# Autodesk Inventor assembly: Gantry1
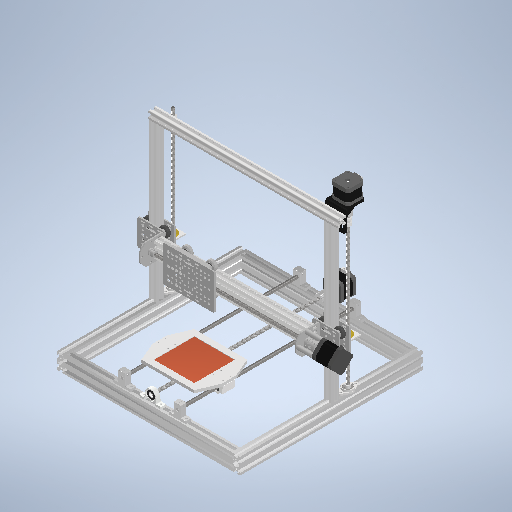
[picture p0: Inventor's stored thumbnail of the model, 512x512]
Saved by Autodesk Inventor 2025.2 (Build 292293000, 293)
## iProperties
Created: 2025-05-31
Part Number: Gantry1
Document SubType Name: Assembly
Designer: Simon
Author: Simon
## Documents named in this file (35)
- C:\Users\Simon\Projects\Hydrogel-3D-Printer\Hardware\Bioprinter Machine Design\Gantry Concept 1\Gantry1.iam
- C:\Users\Simon\Projects\Hydrogel-3D-Printer\Hardware\Bioprinter Machine Design\Gantry Concept 1\SteelShaft_444mm.ipt
- C:\Users\Simon\Projects\Hydrogel-3D-Printer\Hardware\Bioprinter Machine Design\PartsFolder\SK8_LinearShaftSupport.ipt
- C:\Users\Simon\Projects\Hydrogel-3D-Printer\Hardware\Bioprinter Machine Design\PartsFolder\PeltierTEC1_12706.ipt
- C:\Users\Simon\Projects\Hydrogel-3D-Printer\Hardware\Bioprinter Machine Design\PartsFolder\SC8UU\SC8UU.iam
- C:\Users\Simon\Projects\Hydrogel-3D-Printer\Hardware\Bioprinter Machine Design\Gantry Concept 1\BedPlate.ipt
- C:\Users\Simon\Projects\Hydrogel-3D-Printer\Hardware\Bioprinter Machine Design\Gantry Concept 1\BedHousingFrame.ipt
- C:\Users\Simon\Projects\Hydrogel-3D-Printer\Hardware\Bioprinter Machine Design\Gantry Concept 1\2040_AluminimProfile_450.ipt
- C:\Users\Simon\Projects\Hydrogel-3D-Printer\Hardware\Bioprinter Machine Design\Gantry Concept 1\2040_AluminimProfile_410.ipt
- C:\Users\Simon\Projects\Hydrogel-3D-Printer\Hardware\Bioprinter Machine Design\PartsFolder\bracket nema 17.ipt
- C:\Users\Simon\Projects\Hydrogel-3D-Printer\Hardware\Bioprinter Machine Design\Gantry Concept 1\2020_AluminiumProfile_380.ipt
- C:\Users\Simon\Projects\Hydrogel-3D-Printer\Hardware\Bioprinter Machine Design\PartsFolder\Pillow Block Bearing 1\Zinc Alloy Pillow Block Flange Bearing KFL08 ID-8mm.iam
- C:\Users\Simon\Projects\Hydrogel-3D-Printer\Hardware\Bioprinter Machine Design\Gantry Concept 1\TR8x8-4_LeadScrew_385mm.ipt
- C:\Users\Simon\Projects\Hydrogel-3D-Printer\Hardware\Bioprinter Machine Design\PartsFolder\Stepper_17HS4401.ipt
- C:\Users\Simon\Projects\Hydrogel-3D-Printer\Hardware\Bioprinter Machine Design\PartsFolder\GT2_20T_8.ipt
- C:\Users\Simon\Projects\Hydrogel-3D-Printer\Hardware\Bioprinter Machine Design\PartsFolder\Flexible Coupling 5,8.ipt
- C:\Users\Simon\Projects\Hydrogel-3D-Printer\Hardware\Bioprinter Machine Design\Gantry Concept 1\2020_AluminiumProfile_465.ipt
- C:\Users\Simon\Projects\Hydrogel-3D-Printer\Hardware\Bioprinter Machine Design\PartsFolder\TR8x8-4_Nut.ipt
- C:\Users\Simon\Projects\Hydrogel-3D-Printer\Hardware\Bioprinter Machine Design\PartsFolder\Carriage Plate v1.ipt
- C:\Users\Simon\Projects\Hydrogel-3D-Printer\Hardware\Bioprinter Machine Design\PartsFolder\Spacer v2.ipt
- C:\Users\Simon\Projects\Hydrogel-3D-Printer\Hardware\Bioprinter Machine Design\PartsFolder\POM Wheel v2.ipt
- C:\Users\Simon\Projects\Hydrogel-3D-Printer\Hardware\Bioprinter Machine Design\Gantry Concept 1\Lead Screw Driven Actuator (Horizontal)\2040 Al Extrusion - Upper Middle Part (380mm).ipt
- C:\Users\Simon\Projects\Hydrogel-3D-Printer\Hardware\Bioprinter Machine Design\Gantry Concept 1\Lead Screw Driven Actuator (Horizontal)\Threaded Rod Plate Nema 17.ipt
- C:\Users\Simon\Projects\Hydrogel-3D-Printer\Hardware\Bioprinter Machine Design\Gantry Concept 1\Lead Screw Driven Actuator (Horizontal)\Nema 17 Stepper Motor.ipt
- C:\Users\Simon\Projects\Hydrogel-3D-Printer\Hardware\Bioprinter Machine Design\Gantry Concept 1\Lead Screw Driven Actuator (Horizontal)\Aluminum Spacer 1.5in.ipt
- C:\Users\Simon\Projects\Hydrogel-3D-Printer\Hardware\Bioprinter Machine Design\Gantry Concept 1\Lead Screw Driven Actuator (Horizontal)\Flexible Coupling 5mm x 8mm.ipt
- C:\Users\Simon\Projects\Hydrogel-3D-Printer\Hardware\Bioprinter Machine Design\Gantry Concept 1\Lead Screw Driven Actuator (Horizontal)\Lead Screw D8-P2-L400 (ACME).ipt
- C:\Users\Simon\Projects\Hydrogel-3D-Printer\Hardware\Bioprinter Machine Design\Gantry Concept 1\Lead Screw Driven Actuator (Horizontal)\Lead Screw Accessories\Ball Bearing 8 x 16 x 5.ipt
- C:\Users\Simon\Projects\Hydrogel-3D-Printer\Hardware\Bioprinter Machine Design\Gantry Concept 1\Lead Screw Driven Actuator (Horizontal)\Lead Screw Accessories\Lock Collar 8mm.ipt
- C:\Users\Simon\Projects\Hydrogel-3D-Printer\Hardware\Bioprinter Machine Design\Gantry Concept 1\Lead Screw Driven Actuator (Horizontal)\Lead Screw Accessories\Shim Washer 8mm.ipt
- C:\Users\Simon\Projects\Hydrogel-3D-Printer\Hardware\Bioprinter Machine Design\Gantry Concept 1\Lead Screw Driven Actuator (Horizontal)\V-Slot Gantry Kit Universal (for lead screw setup)\Gantry Kit (Horizontal).iam
- C:\Users\Simon\Projects\Hydrogel-3D-Printer\Hardware\Bioprinter Machine Design\Gantry Concept 1\Leadnut Attachment.ipt
- C:\Users\Simon\Projects\Hydrogel-3D-Printer\Hardware\Bioprinter Machine Design\PartsFolder\Pillow Block Bearing 2\KP08_2.iam
- C:\Users\Simon\Projects\Hydrogel-3D-Printer\Hardware\Bioprinter Machine Design\PartsFolder\Nema 17 Flat Mount.ipt
- C:\Users\Simon\Projects\Hydrogel-3D-Printer\Hardware\Bioprinter Machine Design\Gantry Concept 1\TR8x8-4_LeadScrew_420.ipt
## Components (80 placed, 34 different names)
1. SteelShaft_444mm:1 — Mate:1, Mate:3, Flush:1, Flush:4, Mate:5
2. SteelShaft_444mm:2 — Mate:2, Mate:4, Flush:2, Flush:3, Mate:6
3. SK8_LinearShaftSupport:1 — Mate:1, Flush:1, Flush:5, Flush:6, Mate:26
4. SK8_LinearShaftSupport:2 — Mate:2, Flush:2, Flush:5, Flush:6, Mate:23, Flush:19, Flush:45, Flush:47
5. SK8_LinearShaftSupport:3 — Mate:3, Flush:4, Mate:25
6. SK8_LinearShaftSupport:4 — Mate:4, Flush:3, Mate:24
7. PeltierTEC1_12706:1 — Mate:7, Flush:7, Flush:8
8. SC8UU:1 [sub-assembly] — Mate:5, Mate:11, Flush:9, Flush:11, Flush:12
9. SC8UU:2 [sub-assembly] — Mate:6, Flush:10, Mate:12, Flush:11
10. BedPlate:1 — Mate:7, Flush:7, Flush:8, Mate:8, Mate:9, Mate:10
11. BedHousingFrame:1 — Mate:8, Mate:9, Mate:10, Mate:11, Flush:9, Flush:10, Mate:12, Flush:12
12. 2040_AluminimProfile_450:1 — Mate:17, Flush:13, Flush:14, Mate:19, Flush:17, Flush:18, Mate:21, Mate:27, Flush:21, Mate:30, Mate:32
13. 2040_AluminimProfile_450:2 — Mate:18, Flush:15, Flush:16, Mate:23, Mate:24, Mate:28, Flush:20, Mate:29, Mate:31, Flush:45, Flush:46, Flush:48
14. 2040_AluminimProfile_410:1 — Mate:17, Flush:13, Flush:14, Mate:18, Flush:15, Flush:16, Mate:20, Mate:26, Flush:19, Mate:165
15. 2040_AluminimProfile_410:2 — Mate:19, Flush:17, Flush:18, Mate:22, Mate:25, Mate:167, Angle:3
16. bracket nema 17:1 — Mate:36, Mate:37, Mate:40, Angle:1
17. 2020_AluminiumProfile_380:1 — Mate:28, Flush:20, Flush:22, Flush:33, Flush:34, Flush:46
18. 2020_AluminiumProfile_380:2 — Mate:27, Flush:21, Flush:22, Mate:35, Flush:25, Flush:26, Flush:31, Flush:32
19. Zinc Alloy Pillow Block Flange Bearing KFL08 ID-8mm:1 [sub-assembly] — Mate:29, Mate:31, Flush:23, Mate:33, Flush:28
20. Zinc Alloy Pillow Block Flange Bearing KFL08 ID-8mm:2 [sub-assembly] — Mate:30, Mate:32, Flush:23, Mate:34
21. TR8x8-4_LeadScrew_385mm:1 — Mate:33, Flush:24, Mate:36, Mate:38, Flush:28, Mate:41, Mate:42, Mate:45
22. TR8x8-4_LeadScrew_385mm:2 — Mate:34, Flush:24, Mate:43, Mate:46
23. Stepper_17HS4401:1 — Mate:38, Mate:39, Flush:27, Mate:40, Mate:41, Angle:1
24. GT2_20T_8:1 — Mate:42, Flush:29, Mate:44
25. GT2_20T_8:2 — Mate:43, Flush:29
26. Flexible Coupling 5,8:1 — Mate:39, Flush:27, Mate:44
27. 2020_AluminiumProfile_465:1 — Mate:35, Flush:25, Flush:26, Mate:37
28. TR8x8-4_Nut:1 — Mate:45, Flush:30, Mate:164
29. TR8x8-4_Nut:2 — Mate:46, Flush:30
30. Carriage Plate v1:1 — Mate:71, Mate:72, Mate:73, Mate:158, Mate:159, Mate:160
31. Carriage Plate v1:2 — Mate:47, Mate:48, Mate:49, Mate:50, Mate:51, Mate:52, Mate:53, Mate:54, Flush:32, Flush:35, Mate:157, Flush:43, Flush:44
32. Spacer v2:1 — Mate:49, Mate:54, Mate:58, Mate:66
33. Spacer v2:2 — Mate:47, Mate:51, Mate:56, Mate:64
34. Spacer v2:3 — Mate:50, Mate:53, Mate:57, Mate:65
35. Spacer v2:4 — Mate:48, Mate:52, Mate:55, Mate:63
36. Spacer v2:5 — Mate:59, Mate:67
37. Spacer v2:6 — Mate:61, Mate:68, Mate:71
38. Spacer v2:7 — Mate:62, Mate:69
39. Spacer v2:8 — Mate:60, Mate:70, Mate:72, Mate:73
40. POM Wheel v2:1 — Mate:58, Mate:60, Mate:66, Mate:70
41. POM Wheel v2:2 — Mate:57, Mate:62, Mate:65, Mate:69
42. POM Wheel v2:3 — Mate:56, Mate:59, Mate:64, Mate:67
43. POM Wheel v2:4 — Mate:55, Mate:61, Mate:63, Mate:68, Flush:31
44. Carriage Plate v1:5 — Mate:161, Mate:162, Mate:163
45. Carriage Plate v1:6 — Flush:34, Flush:35
46. Spacer v2:17
47. Spacer v2:18
48. Spacer v2:19
49. Spacer v2:20
50. Spacer v2:21
51. Spacer v2:22
52. Spacer v2:23
53. Spacer v2:24
54. POM Wheel v2:9
55. POM Wheel v2:10
56. POM Wheel v2:11 — Flush:33
57. POM Wheel v2:12
58. 2040 Al Extrusion - Upper Middle Part (380mm):1
59. Threaded Rod Plate Nema 17:1 — Mate:157, Flush:43, Flush:44
60. Threaded Rod Plate Nema 17:2
61. Nema 17 Stepper Motor:1
62. Aluminum Spacer 1.5in:1
63. Aluminum Spacer 1.5in:2
64. Aluminum Spacer 1.5in:3
65. Flexible Coupling 5mm x 8mm:1
66. Lead Screw D8-P2-L400 (ACME):1
67. Ball Bearing 8 x 16 x 5:1
68. Ball Bearing 8 x 16 x 5:2
69. Lock Collar 8mm:1
70. Lock Collar 8mm:2
71. Shim Washer 8mm:1
72. Shim Washer 8mm:2
73. Gantry Kit (Horizontal):1 [sub-assembly]
74. Leadnut Attachment:1 — Mate:158, Mate:159, Mate:160
75. Leadnut Attachment:2 — Mate:161, Mate:162, Mate:163, Mate:164
76. Stepper_17HS4401:2 — Mate:168, Angle:2, Mate:169, Mate:170, Flush:49, Mate:172
77. KP08_2:1 [sub-assembly] — Mate:165, Flush:47, Flush:48, Mate:166
78. Nema 17 Flat Mount:1 — Mate:166, Mate:167, Mate:168, Angle:2, Angle:3, Mate:169
79. Flexible Coupling 5,8:2 — Mate:170, Flush:49, Mate:171
80. TR8x8-4_LeadScrew_420:1 — Mate:171, Mate:172
## Relationships (194: Mate 141, Flush 49, Angle 3, RelateRotateTranslate 1)
- Mate:1: SteelShaft_444mm:1 ↔ SK8_LinearShaftSupport:1
- Mate:2: SteelShaft_444mm:2 ↔ SK8_LinearShaftSupport:2
- Mate:3: SteelShaft_444mm:1 ↔ SK8_LinearShaftSupport:3
- Mate:4: SteelShaft_444mm:2 ↔ SK8_LinearShaftSupport:4
- Flush:1: SteelShaft_444mm:1 ↔ SK8_LinearShaftSupport:1
- Flush:2: SteelShaft_444mm:2 ↔ SK8_LinearShaftSupport:2
- Flush:3: SteelShaft_444mm:2 ↔ SK8_LinearShaftSupport:4
- Flush:4: SteelShaft_444mm:1 ↔ SK8_LinearShaftSupport:3
- Flush:5: SK8_LinearShaftSupport:1 ↔ SK8_LinearShaftSupport:2
- Flush:6: SK8_LinearShaftSupport:1 ↔ SK8_LinearShaftSupport:2
- Mate:5: SteelShaft_444mm:1 ↔ SC8UU:1
- Mate:6: SteelShaft_444mm:2 ↔ SC8UU:2
- Mate:7: PeltierTEC1_12706:1 ↔ BedPlate:1
- Flush:7 (-30 mm): PeltierTEC1_12706:1 ↔ BedPlate:1
- Flush:8 (30 mm): PeltierTEC1_12706:1 ↔ BedPlate:1
- Mate:8: BedPlate:1 ↔ BedHousingFrame:1
- Mate:9: BedPlate:1 ↔ BedHousingFrame:1
- Mate:10: BedPlate:1 ↔ BedHousingFrame:1
- Mate:11: SC8UU:1 ↔ BedHousingFrame:1
- Flush:9: SC8UU:1 ↔ BedHousingFrame:1
- Flush:10: SC8UU:2 ↔ BedHousingFrame:1
- Mate:12: SC8UU:2 ↔ BedHousingFrame:1
- Flush:11: SC8UU:1 ↔ SC8UU:2
- Flush:12 (50 mm): SC8UU:1 ↔ BedHousingFrame:1
- Mate:17: 2040_AluminimProfile_450:1 ↔ 2040_AluminimProfile_410:1
- Flush:13: 2040_AluminimProfile_450:1 ↔ 2040_AluminimProfile_410:1
- Flush:14: 2040_AluminimProfile_450:1 ↔ 2040_AluminimProfile_410:1
- Mate:18: 2040_AluminimProfile_450:2 ↔ 2040_AluminimProfile_410:1
- Flush:15: 2040_AluminimProfile_450:2 ↔ 2040_AluminimProfile_410:1
- Flush:16: 2040_AluminimProfile_450:2 ↔ 2040_AluminimProfile_410:1
- Mate:19: 2040_AluminimProfile_450:1 ↔ 2040_AluminimProfile_410:2
- Flush:17: 2040_AluminimProfile_450:1 ↔ 2040_AluminimProfile_410:2
- Flush:18: 2040_AluminimProfile_450:1 ↔ 2040_AluminimProfile_410:2
- Mate:20: 2040_AluminimProfile_410:1
- Mate:21: 2040_AluminimProfile_450:1
- Mate:22: 2040_AluminimProfile_410:2
- Mate:23: SK8_LinearShaftSupport:2 ↔ 2040_AluminimProfile_450:2
- Mate:24: SK8_LinearShaftSupport:4 ↔ 2040_AluminimProfile_450:2
- Mate:25: SK8_LinearShaftSupport:3 ↔ 2040_AluminimProfile_410:2
- Mate:26: SK8_LinearShaftSupport:1 ↔ 2040_AluminimProfile_410:1
- Flush:19 (3 mm): SK8_LinearShaftSupport:2 ↔ 2040_AluminimProfile_410:1
- Mate:27: 2040_AluminimProfile_450:1 ↔ 2020_AluminiumProfile_380:2
- Mate:28: 2040_AluminimProfile_450:2 ↔ 2020_AluminiumProfile_380:1
- Flush:20: 2040_AluminimProfile_450:2 ↔ 2020_AluminiumProfile_380:1
- Flush:21: 2040_AluminimProfile_450:1 ↔ 2020_AluminiumProfile_380:2
- Flush:22: 2020_AluminiumProfile_380:1 ↔ 2020_AluminiumProfile_380:2
- Mate:29: 2040_AluminimProfile_450:2 ↔ Zinc Alloy Pillow Block Flange Bearing KFL08 ID-8mm:1
- Mate:30: 2040_AluminimProfile_450:1 ↔ Zinc Alloy Pillow Block Flange Bearing KFL08 ID-8mm:2
- Mate:31: 2040_AluminimProfile_450:2 ↔ Zinc Alloy Pillow Block Flange Bearing KFL08 ID-8mm:1
- Mate:32: 2040_AluminimProfile_450:1 ↔ Zinc Alloy Pillow Block Flange Bearing KFL08 ID-8mm:2
- Flush:23: Zinc Alloy Pillow Block Flange Bearing KFL08 ID-8mm:1 ↔ Zinc Alloy Pillow Block Flange Bearing KFL08 ID-8mm:2
- Mate:33: Zinc Alloy Pillow Block Flange Bearing KFL08 ID-8mm:1 ↔ TR8x8-4_LeadScrew_385mm:1
- Mate:34: Zinc Alloy Pillow Block Flange Bearing KFL08 ID-8mm:2 ↔ TR8x8-4_LeadScrew_385mm:2
- Flush:24: TR8x8-4_LeadScrew_385mm:1 ↔ TR8x8-4_LeadScrew_385mm:2
- Mate:35: 2020_AluminiumProfile_380:2 ↔ 2020_AluminiumProfile_465:1
- Flush:25: 2020_AluminiumProfile_380:2 ↔ 2020_AluminiumProfile_465:1
- Flush:26: 2020_AluminiumProfile_380:2 ↔ 2020_AluminiumProfile_465:1
- Mate:36: bracket nema 17:1 ↔ TR8x8-4_LeadScrew_385mm:1
- Mate:37: bracket nema 17:1 ↔ 2020_AluminiumProfile_465:1
- Mate:38: TR8x8-4_LeadScrew_385mm:1 ↔ Stepper_17HS4401:1
- Mate:39: Stepper_17HS4401:1 ↔ Flexible Coupling 5,8:1
- Flush:27 (5 mm): Stepper_17HS4401:1 ↔ Flexible Coupling 5,8:1
- Mate:40: bracket nema 17:1 ↔ Stepper_17HS4401:1
- Flush:28: Zinc Alloy Pillow Block Flange Bearing KFL08 ID-8mm:1 ↔ TR8x8-4_LeadScrew_385mm:1
- Mate:41: TR8x8-4_LeadScrew_385mm:1 ↔ Stepper_17HS4401:1
- Angle:1 (0 deg): bracket nema 17:1 ↔ Stepper_17HS4401:1
- Mate:42: TR8x8-4_LeadScrew_385mm:1 ↔ GT2_20T_8:1
- Mate:43: TR8x8-4_LeadScrew_385mm:2 ↔ GT2_20T_8:2
- Flush:29: GT2_20T_8:1 ↔ GT2_20T_8:2
- Mate:44 (5 mm): GT2_20T_8:1 ↔ Flexible Coupling 5,8:1
- Mate:45: TR8x8-4_LeadScrew_385mm:1 ↔ TR8x8-4_Nut:1
- Mate:46: TR8x8-4_LeadScrew_385mm:2 ↔ TR8x8-4_Nut:2
- Flush:30: TR8x8-4_Nut:1 ↔ TR8x8-4_Nut:2
- Mate:47: Carriage Plate v1:2 ↔ Spacer v2:2
- Mate:48: Carriage Plate v1:2 ↔ Spacer v2:4
- Mate:49: Carriage Plate v1:2 ↔ Spacer v2:1
- Mate:50: Carriage Plate v1:2 ↔ Spacer v2:3
- Mate:51: Carriage Plate v1:2 ↔ Spacer v2:2
- Mate:52: Carriage Plate v1:2 ↔ Spacer v2:4
- Mate:53: Carriage Plate v1:2 ↔ Spacer v2:3
- Mate:54: Carriage Plate v1:2 ↔ Spacer v2:1
- Mate:55: Spacer v2:4 ↔ POM Wheel v2:4
- Mate:56: Spacer v2:2 ↔ POM Wheel v2:3
- Mate:57: Spacer v2:3 ↔ POM Wheel v2:2
- Mate:58: Spacer v2:1 ↔ POM Wheel v2:1
- Mate:59: Spacer v2:5 ↔ POM Wheel v2:3
- Mate:60: Spacer v2:8 ↔ POM Wheel v2:1
- Mate:61: Spacer v2:6 ↔ POM Wheel v2:4
- Mate:62: Spacer v2:7 ↔ POM Wheel v2:2
- Mate:63: Spacer v2:4 ↔ POM Wheel v2:4
- Mate:64: Spacer v2:2 ↔ POM Wheel v2:3
- Mate:65: Spacer v2:3 ↔ POM Wheel v2:2
- Mate:66: Spacer v2:1 ↔ POM Wheel v2:1
- Mate:67: Spacer v2:5 ↔ POM Wheel v2:3
- Mate:68: Spacer v2:6 ↔ POM Wheel v2:4
- Mate:69: Spacer v2:7 ↔ POM Wheel v2:2
- Mate:70: Spacer v2:8 ↔ POM Wheel v2:1
- Mate:71: Carriage Plate v1:1 ↔ Spacer v2:6
- Mate:72: Carriage Plate v1:1 ↔ Spacer v2:8
- Mate:73: Carriage Plate v1:1 ↔ Spacer v2:8
- Flush:31: 2020_AluminiumProfile_380:2 ↔ POM Wheel v2:4
- Flush:32: 2020_AluminiumProfile_380:2 ↔ Carriage Plate v1:2
- [Mate]: Carriage Plate v1:6 ↔ Spacer v2:18
- [Mate]: Carriage Plate v1:6 ↔ Spacer v2:20
- [Mate]: Carriage Plate v1:6 ↔ Spacer v2:17
- [Mate]: Carriage Plate v1:6 ↔ Spacer v2:19
- [Mate]: Carriage Plate v1:6 ↔ Spacer v2:18
- [Mate]: Carriage Plate v1:6 ↔ Spacer v2:20
- [Mate]: Carriage Plate v1:6 ↔ Spacer v2:19
- [Mate]: Carriage Plate v1:6 ↔ Spacer v2:17
- [Mate]: Spacer v2:20 ↔ POM Wheel v2:12
- [Mate]: Spacer v2:18 ↔ POM Wheel v2:11
- [Mate]: Spacer v2:19 ↔ POM Wheel v2:10
- [Mate]: Spacer v2:17 ↔ POM Wheel v2:9
- [Mate]: Spacer v2:21 ↔ POM Wheel v2:11
- [Mate]: Spacer v2:24 ↔ POM Wheel v2:9
- [Mate]: Spacer v2:22 ↔ POM Wheel v2:12
- [Mate]: Spacer v2:23 ↔ POM Wheel v2:10
- [Mate]: Spacer v2:20 ↔ POM Wheel v2:12
- [Mate]: Spacer v2:18 ↔ POM Wheel v2:11
- [Mate]: Spacer v2:19 ↔ POM Wheel v2:10
- [Mate]: Spacer v2:17 ↔ POM Wheel v2:9
- [Mate]: Spacer v2:21 ↔ POM Wheel v2:11
- [Mate]: Spacer v2:22 ↔ POM Wheel v2:12
- [Mate]: Spacer v2:23 ↔ POM Wheel v2:10
- [Mate]: Spacer v2:24 ↔ POM Wheel v2:9
- [Mate]: Carriage Plate v1:5 ↔ Spacer v2:22
- [Mate]: Carriage Plate v1:5 ↔ Spacer v2:24
- [Mate]: Carriage Plate v1:5 ↔ Spacer v2:24
- Flush:33: 2020_AluminiumProfile_380:1 ↔ POM Wheel v2:11
- Flush:34: 2020_AluminiumProfile_380:1 ↔ Carriage Plate v1:6
- Flush:35: Carriage Plate v1:2 ↔ Carriage Plate v1:6
- [Mate]: 2040 Al Extrusion - Upper Middle Part (380mm):1 ↔ Threaded Rod Plate Nema 17:1
- [Mate]: 2040 Al Extrusion - Upper Middle Part (380mm):1 ↔ Threaded Rod Plate Nema 17:2
- [Flush] (-4 mm): 2040 Al Extrusion - Upper Middle Part (380mm):1 ↔ Threaded Rod Plate Nema 17:2
- [Flush]: Threaded Rod Plate Nema 17:1 ↔ Threaded Rod Plate Nema 17:2
- [Flush]: Threaded Rod Plate Nema 17:1 ↔ Threaded Rod Plate Nema 17:2
- [Flush] (-6.5 mm): 2040 Al Extrusion - Upper Middle Part (380mm):1 ↔ Threaded Rod Plate Nema 17:2
- [Mate]: Threaded Rod Plate Nema 17:2 ↔ Aluminum Spacer 1.5in:2
- [Mate]: Threaded Rod Plate Nema 17:2 ↔ Aluminum Spacer 1.5in:1
- [Mate]: Threaded Rod Plate Nema 17:2 ↔ Aluminum Spacer 1.5in:3
- [Mate]: Threaded Rod Plate Nema 17:2 ↔ Aluminum Spacer 1.5in:2
- [Mate]: Threaded Rod Plate Nema 17:2 ↔ Aluminum Spacer 1.5in:1
- [Mate]: Threaded Rod Plate Nema 17:2 ↔ Aluminum Spacer 1.5in:3
- [Mate]: Nema 17 Stepper Motor:1 ↔ Aluminum Spacer 1.5in:1
- [Mate]: Nema 17 Stepper Motor:1 ↔ Aluminum Spacer 1.5in:2
- [Mate]: Nema 17 Stepper Motor:1 ↔ Aluminum Spacer 1.5in:3
- [Mate]: Nema 17 Stepper Motor:1 ↔ Flexible Coupling 5mm x 8mm:1
- [Flush]: Nema 17 Stepper Motor:1 ↔ Flexible Coupling 5mm x 8mm:1
- [Mate]: Threaded Rod Plate Nema 17:1 ↔ Lead Screw D8-P2-L400 (ACME):1
- [Mate]: Flexible Coupling 5mm x 8mm:1 ↔ Lead Screw D8-P2-L400 (ACME):1
- [Mate]: Threaded Rod Plate Nema 17:1 ↔ Ball Bearing 8 x 16 x 5:1
- [Mate]: Threaded Rod Plate Nema 17:2 ↔ Ball Bearing 8 x 16 x 5:2
- [Mate]: Threaded Rod Plate Nema 17:1 ↔ Ball Bearing 8 x 16 x 5:1
- [Mate]: Threaded Rod Plate Nema 17:2 ↔ Ball Bearing 8 x 16 x 5:2
- [Mate]: Lead Screw D8-P2-L400 (ACME):1 ↔ Lock Collar 8mm:1
- [Mate]: Lead Screw D8-P2-L400 (ACME):1 ↔ Lock Collar 8mm:2
- [Mate]: Lead Screw D8-P2-L400 (ACME):1 ↔ Shim Washer 8mm:1
- [Mate]: Lead Screw D8-P2-L400 (ACME):1 ↔ Shim Washer 8mm:2
- [Mate]: Ball Bearing 8 x 16 x 5:2 ↔ Shim Washer 8mm:2
- [Mate]: Ball Bearing 8 x 16 x 5:1 ↔ Shim Washer 8mm:1
- [Mate]: Lock Collar 8mm:1 ↔ Shim Washer 8mm:1
- [Mate]: Lock Collar 8mm:2 ↔ Shim Washer 8mm:2
- [Mate]: Lead Screw D8-P2-L400 (ACME):1 ↔ Lock Collar 8mm:1
- [Mate]: Lead Screw D8-P2-L400 (ACME):1 ↔ Lock Collar 8mm:2
- [Flush]: Flexible Coupling 5mm x 8mm:1 ↔ Lead Screw D8-P2-L400 (ACME):1
- [Mate]: Lead Screw D8-P2-L400 (ACME):1 ↔ Gantry Kit (Horizontal):1
- [Flush]: Threaded Rod Plate Nema 17:1 ↔ Gantry Kit (Horizontal):1
- [RelateRotateTranslate] (25.133 mm): Lead Screw D8-P2-L400 (ACME):1 ↔ Gantry Kit (Horizontal):1
- Mate:157: Carriage Plate v1:2 ↔ Threaded Rod Plate Nema 17:1
- Flush:43: Carriage Plate v1:2 ↔ Threaded Rod Plate Nema 17:1
- Flush:44: Carriage Plate v1:2 ↔ Threaded Rod Plate Nema 17:1
- Flush:45 (136 mm): SK8_LinearShaftSupport:2 ↔ 2040_AluminimProfile_450:2
- Flush:46 (225 mm): 2040_AluminimProfile_450:2 ↔ 2020_AluminiumProfile_380:1
- Mate:158: Carriage Plate v1:1 ↔ Leadnut Attachment:1
- Mate:159: Carriage Plate v1:1 ↔ Leadnut Attachment:1
- Mate:160: Carriage Plate v1:1 ↔ Leadnut Attachment:1
- Mate:161: Carriage Plate v1:5 ↔ Leadnut Attachment:2
- Mate:162: Carriage Plate v1:5 ↔ Leadnut Attachment:2
- Mate:163: Carriage Plate v1:5 ↔ Leadnut Attachment:2
- Mate:164: TR8x8-4_Nut:1 ↔ Leadnut Attachment:2
- Mate:165: 2040_AluminimProfile_410:1 ↔ KP08_2:1
- Flush:47: SK8_LinearShaftSupport:2 ↔ KP08_2:1
- Flush:48 (197.5 mm): 2040_AluminimProfile_450:2 ↔ KP08_2:1
- Mate:166: KP08_2:1 ↔ Nema 17 Flat Mount:1
- Mate:167: 2040_AluminimProfile_410:2 ↔ Nema 17 Flat Mount:1
- Mate:168: Stepper_17HS4401:2 ↔ Nema 17 Flat Mount:1
- Angle:2 (0 deg): Stepper_17HS4401:2 ↔ Nema 17 Flat Mount:1
- Angle:3 (0 deg): 2040_AluminimProfile_410:2 ↔ Nema 17 Flat Mount:1
- Mate:169: Stepper_17HS4401:2 ↔ Nema 17 Flat Mount:1
- Mate:170: Stepper_17HS4401:2 ↔ Flexible Coupling 5,8:2
- Flush:49 (5 mm): Stepper_17HS4401:2 ↔ Flexible Coupling 5,8:2
- Mate:171: Flexible Coupling 5,8:2 ↔ TR8x8-4_LeadScrew_420:1
- Mate:172: Stepper_17HS4401:2 ↔ TR8x8-4_LeadScrew_420:1
## Named parameters: d134_d78 = 0 mm, d135_d79 = 0 mm, d136_d80 = 0 mm, d137_d81 = 0 mm, d138_d82 = 0 mm, d139_d83 = 0 mm, d140_d84 = 0 mm, d141_d85 = 0 mm, d142_d102 = 0 mm, d143_d103 = 0 mm, d144_d104 = 0 mm, d145_d86 = 0 mm, d146_d87 = 0 mm, d147_d88 = 0 mm, d148_d89 = 0 mm, d149_d90 = 0 mm, d150_d91 = 0 mm, d151_d92 = 0 mm, d152_d93 = 0 mm, d153_d94 = 0 mm, d154_d95 = 0 mm, d155_d96 = 0 mm, d156_d97 = 0 mm, d157_d98 = 0 mm, d158_d99 = 0 mm, d159_d100 = 0 mm, d160_d101 = 0 mm, d165_d26 = 0 mm, d166_d27 = -4 mm, d167_d28 = 0 mm, d168_d29 = 0 mm, d169_d30 = -6.5 mm, d170_d31 = 0 mm, d171_d32 = 0 mm, d172_d33 = 0 mm, d173_d34 = 0 mm, d174_d35 = 0 mm, d175_d36 = 0 mm, d176_d37 = 0 mm, d177_d38 = 0 mm, d178_d39 = 0 mm, d179_d40 = 0 mm, d180_d41 = 0 mm, d181_d42 = 0 mm, d182_d43 = 0 mm, d183_d44 = 0 mm, d184_d45 = 0 mm, d185_d46 = 0 mm, d186_d47 = 0 mm, d187_d48 = 0 mm, d188_d49 = 0 mm, d189_d50 = 0 mm, d190_d51 = 0 mm, d191_d52 = 0 mm, d192_d53 = 0 mm, d193_d54 = 0 mm, d194_d55 = 0 mm, d195_d56 = 0 mm, d196_d57 = 0 mm, d197_d58 = 0 mm, d198_d59 = 0 mm, d199_d60 = 0 mm, d200_d61 = 25.133 mm
